# Autodesk Inventor assembly: am-3322+RhinoTrackDriveModule_MIR14
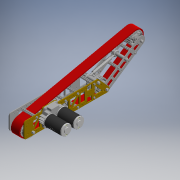
[picture p0: Inventor's stored thumbnail of the model, 180x180]
Saved by Autodesk Inventor 2016 SP1 (Build 200210100, 210)
## iProperties
Created: 2015-12-17
Part Number: am-3322+RhinoTrackDriveModule_MIR14
Description: STEP AP203
Document SubType Name: Assembly
Designer: steele
Mass: 4285.93 g
Surface Area: 10743.9 cm^2
Volume: 2788.38 cm^3
Density: 1.53707 g/cm^3
Title: am-3322 Rhino Track Drive Module.STEP
Revision Number: ANY
Sending System: SolidWorks 2014
Preprocessor: SwSTEP 2.0
## Documents named in this file (29)
- C:\snobotics\CAD-Development\robSteele\SnoBotics2016\RhinoTrackDriveModule\am-3322+RhinoTrackDriveModule_MIR14.iam
- C:\snobotics\CAD-Development\robSteele\SnoBotics2016\RhinoTrackDriveModule\am-3319 Inside Plate_MIR14.ipt
- C:\snobotics\CAD-Development\robSteele\SnoBotics2016\RhinoTrackDriveModule\20T pulley back to back_MIR14.iam
- C:\snobotics\CAD-Development\robSteele\SnoBotics2016\RhinoTrackDriveModule\am-1393 375 washer_MIR14.ipt
- C:\snobotics\CAD-Development\robSteele\SnoBotics2016\RhinoTrackDriveModule\am-3320 Upper Bar_MIR14.ipt
- C:\snobotics\CAD-Development\robSteele\SnoBotics2016\RhinoTrackDriveModule\Track Belt_MIR14.ipt
- C:\snobotics\CAD-Development\robSteele\SnoBotics2016\RhinoTrackDriveModule\am-2598_107 2016 KOP Toughbox Mini_MIR14.iam
- C:\snobotics\CAD-Development\robSteele\SnoBotics2016\RhinoTrackDriveModule\am-3318 Outside Plate_MIR14.ipt
- C:\snobotics\CAD-Development\robSteele\SnoBotics2016\RhinoTrackDriveModule\FR8ZZ Hex Bearing_MIR14.ipt
- C:\snobotics\CAD-Development\robSteele\SnoBotics2016\RhinoTrackDriveModule\am-0207a 250 Sprocket and Pulley Spacer_MIR14.ipt
- C:\snobotics\CAD-Development\robSteele\SnoBotics2016\RhinoTrackDriveModule\10-24 Hex Washer Rolling x 1.25_93882A213_MIR14.ipt
- C:\snobotics\CAD-Development\robSteele\SnoBotics2016\RhinoTrackDriveModule\425-5M-15_MIR14.ipt
- C:\snobotics\CAD-Development\robSteele\SnoBotics2016\RhinoTrackDriveModule\500EX Hex Hub_MIR14.ipt
- C:\snobotics\CAD-Development\robSteele\SnoBotics2016\RhinoTrackDriveModule\BHCS 10-32 x 1000_SBHCSCREW 0.19-32x0.5-HX-C_MIR14.ipt
- C:\snobotics\CAD-Development\robSteele\SnoBotics2016\RhinoTrackDriveModule\10-32 Nylock Nut_MIR14.ipt
- C:\snobotics\CAD-Development\robSteele\SnoBotics2016\RhinoTrackDriveModule\0985x0420 PVC Spacer_MIR14.ipt
- C:\snobotics\CAD-Development\robSteele\SnoBotics2016\RhinoTrackDriveModule\Churro 3375_MIR14.ipt
- C:\snobotics\CAD-Development\robSteele\SnoBotics2016\RhinoTrackDriveModule\FHTS 0.25-20-0.75_FHTS 0.25-20-G-0.75-C_MIR14.ipt
- C:\snobotics\CAD-Development\robSteele\SnoBotics2016\RhinoTrackDriveModule\375-16 x 4.25 Hex Bolt_HFBOLT 0.375-16x2.5x1-C_MIR14.ipt
- C:\snobotics\CAD-Development\robSteele\SnoBotics2016\RhinoTrackDriveModule\3-8-16 NyLock Nut - Mcm 95615A140_95615A140_MIR14.ipt
- C:\snobotics\CAD-Development\robSteele\SnoBotics2016\RhinoTrackDriveModule\10-32x0625_shcs_HX-SHCS 0.19-32x1.375x1-C_MIR14.ipt
- C:\snobotics\CAD-Development\robSteele\SnoBotics2016\RhinoTrackDriveModule\187x385 spacer 13RS038518_MIR14.ipt
- C:\snobotics\CAD-Development\robSteele\SnoBotics2016\RhinoTrackDriveModule\am-0243 spacer 1860x0420_MIR14.ipt
- C:\snobotics\CAD-Development\robSteele\SnoBotics2016\RhinoTrackDriveModule\500 Hex Collar Clamp_MIR14.iam
- C:\snobotics\CAD-Development\robSteele\SnoBotics2016\RhinoTrackDriveModule\Spacer am-1181_MIR14.ipt
- C:\snobotics\CAD-Development\robSteele\SnoBotics2016\RhinoTrackDriveModule\Round Collar 375_MIR14.ipt
- C:\snobotics\CAD-Development\robSteele\SnoBotics2016\RhinoTrackDriveModule\am-2243 brass spacer_MIR14.ipt
- C:\snobotics\CAD-Development\robSteele\SnoBotics2016\RhinoTrackDriveModule\am-3321 turnbuckle_MIR14.iam
- C:\snobotics\autodesk\2016\FRC KOP 2016\Motors\MOT_CIM-Motor_217-2000_MIR15.iam
## Components (92 placed, 28 different names)
1. am-3319 Inside Plate_MIR14:1
2. 20T pulley back to back_MIR14:1 [sub-assembly]
3. am-1393 375 washer_MIR14:1
4. am-3320 Upper Bar_MIR14:1
5. am-3320 Upper Bar_MIR14:2
6. 20T pulley back to back_MIR14:2 [sub-assembly]
7. Track Belt_MIR14:1
8. am-2598_107 2016 KOP Toughbox Mini_MIR14:1 [sub-assembly] — Insert:1, Insert:2
9. am-3318 Outside Plate_MIR14:1
10. 20T pulley back to back_MIR14:3 [sub-assembly]
11. 20T pulley back to back_MIR14:4 [sub-assembly]
12. FR8ZZ Hex Bearing_MIR14:1
13. am-0207a 250 Sprocket and Pulley Spacer_MIR14:1
14. 10-24 Hex Washer Rolling x 1.25_93882A213_MIR14:1
15. 10-24 Hex Washer Rolling x 1.25_93882A213_MIR14:2
16. 10-24 Hex Washer Rolling x 1.25_93882A213_MIR14:3
17. 425-5M-15_MIR14:1
18. 500EX Hex Hub_MIR14:1
19. BHCS 10-32 x 1000_SBHCSCREW 0.19-32x0.5-HX-C_MIR14:1
20. BHCS 10-32 x 1000_SBHCSCREW 0.19-32x0.5-HX-C_MIR14:2
21. BHCS 10-32 x 1000_SBHCSCREW 0.19-32x0.5-HX-C_MIR14:3
22. BHCS 10-32 x 1000_SBHCSCREW 0.19-32x0.5-HX-C_MIR14:4
23. BHCS 10-32 x 1000_SBHCSCREW 0.19-32x0.5-HX-C_MIR14:5
24. BHCS 10-32 x 1000_SBHCSCREW 0.19-32x0.5-HX-C_MIR14:6
25. 10-32 Nylock Nut_MIR14:1
26. 10-32 Nylock Nut_MIR14:2
27. 10-32 Nylock Nut_MIR14:3
28. 10-32 Nylock Nut_MIR14:4
29. 10-32 Nylock Nut_MIR14:5
30. 10-32 Nylock Nut_MIR14:6
31. am-1393 375 washer_MIR14:2
32. am-1393 375 washer_MIR14:3
33. 0985x0420 PVC Spacer_MIR14:1
34. 0985x0420 PVC Spacer_MIR14:2
35. Churro 3375_MIR14:1
36. Churro 3375_MIR14:2
37. Churro 3375_MIR14:3
38. Churro 3375_MIR14:4
39. Churro 3375_MIR14:5
40. Churro 3375_MIR14:6
41. Churro 3375_MIR14:7
42. FHTS 0.25-20-0.75_FHTS 0.25-20-G-0.75-C_MIR14:1
43. FHTS 0.25-20-0.75_FHTS 0.25-20-G-0.75-C_MIR14:2
44. FHTS 0.25-20-0.75_FHTS 0.25-20-G-0.75-C_MIR14:3
45. FHTS 0.25-20-0.75_FHTS 0.25-20-G-0.75-C_MIR14:4
46. FHTS 0.25-20-0.75_FHTS 0.25-20-G-0.75-C_MIR14:5
47. FHTS 0.25-20-0.75_FHTS 0.25-20-G-0.75-C_MIR14:6
48. FHTS 0.25-20-0.75_FHTS 0.25-20-G-0.75-C_MIR14:7
49. FHTS 0.25-20-0.75_FHTS 0.25-20-G-0.75-C_MIR14:8
50. FHTS 0.25-20-0.75_FHTS 0.25-20-G-0.75-C_MIR14:9
51. FHTS 0.25-20-0.75_FHTS 0.25-20-G-0.75-C_MIR14:10
52. FHTS 0.25-20-0.75_FHTS 0.25-20-G-0.75-C_MIR14:11
53. FHTS 0.25-20-0.75_FHTS 0.25-20-G-0.75-C_MIR14:12
54. FHTS 0.25-20-0.75_FHTS 0.25-20-G-0.75-C_MIR14:13
55. FHTS 0.25-20-0.75_FHTS 0.25-20-G-0.75-C_MIR14:14
56. 375-16 x 4.25 Hex Bolt_HFBOLT 0.375-16x2.5x1-C_MIR14:1
57. 375-16 x 4.25 Hex Bolt_HFBOLT 0.375-16x2.5x1-C_MIR14:2
58. 375-16 x 4.25 Hex Bolt_HFBOLT 0.375-16x2.5x1-C_MIR14:3
59. 3-8-16 NyLock Nut - Mcm 95615A140_95615A140_MIR14:1
60. 3-8-16 NyLock Nut - Mcm 95615A140_95615A140_MIR14:2
61. 3-8-16 NyLock Nut - Mcm 95615A140_95615A140_MIR14:3
62. 10-32x0625_shcs_HX-SHCS 0.19-32x1.375x1-C_MIR14:1
63. 10-32x0625_shcs_HX-SHCS 0.19-32x1.375x1-C_MIR14:2
64. 10-32x0625_shcs_HX-SHCS 0.19-32x1.375x1-C_MIR14:3
65. 10-32x0625_shcs_HX-SHCS 0.19-32x1.375x1-C_MIR14:4
66. FHTS 0.25-20-0.75_FHTS 0.25-20-G-0.75-C_MIR14:15
67. FHTS 0.25-20-0.75_FHTS 0.25-20-G-0.75-C_MIR14:16
68. FHTS 0.25-20-0.75_FHTS 0.25-20-G-0.75-C_MIR14:17
69. FHTS 0.25-20-0.75_FHTS 0.25-20-G-0.75-C_MIR14:18
70. am-1393 375 washer_MIR14:4
71. 187x385 spacer 13RS038518_MIR14:1
72. 375-16 x 4.25 Hex Bolt_HFBOLT 0.375-16x2.5x1-C_MIR14:4
73. 3-8-16 NyLock Nut - Mcm 95615A140_95615A140_MIR14:4
74. 3-8-16 NyLock Nut - Mcm 95615A140_95615A140_MIR14:5
75. 375-16 x 4.25 Hex Bolt_HFBOLT 0.375-16x2.5x1-C_MIR14:5
76. am-0243 spacer 1860x0420_MIR14:1
77. am-0243 spacer 1860x0420_MIR14:2
78. 500 Hex Collar Clamp_MIR14:1 [sub-assembly]
79. Churro 3375_MIR14:8
80. Churro 3375_MIR14:9
81. 375-16 x 4.25 Hex Bolt_HFBOLT 0.375-16x2.5x1-C_MIR14:6
82. 3-8-16 NyLock Nut - Mcm 95615A140_95615A140_MIR14:6
83. Spacer am-1181_MIR14:1
84. Round Collar 375_MIR14:1
85. Round Collar 375_MIR14:2
86. am-2243 brass spacer_MIR14:1
87. am-2243 brass spacer_MIR14:2
88. am-1393 375 washer_MIR14:5
89. am-1393 375 washer_MIR14:6
90. am-3321 turnbuckle_MIR14:1 [sub-assembly]
91. MOT_CIM-Motor_217-2000_MIR15:1 [sub-assembly] — Insert:1
92. MOT_CIM-Motor_217-2000_MIR15:2 [sub-assembly] — Insert:2
## Relationships (2: Insert 2)
- Insert:1: am-2598_107 2016 KOP Toughbox Mini_MIR14:1 ↔ MOT_CIM-Motor_217-2000_MIR15:1
- Insert:2: am-2598_107 2016 KOP Toughbox Mini_MIR14:1 ↔ MOT_CIM-Motor_217-2000_MIR15:2
